# Autodesk Inventor assembly: Leg_Front+Right
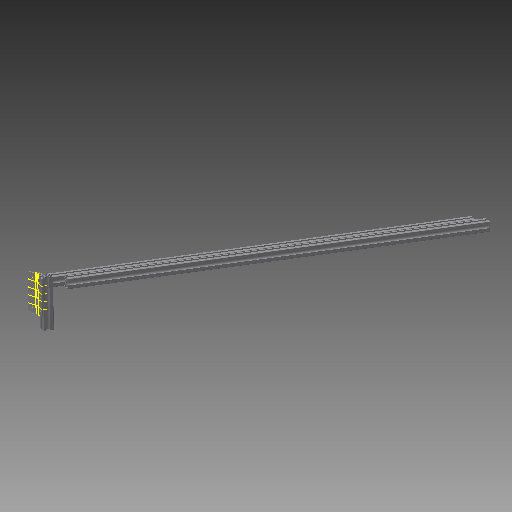
[picture p0: Inventor's stored thumbnail of the model, 512x512]
Saved by Autodesk Inventor 2019 (Build 230136000, 136)
## iProperties
Created: 2019-04-07
Part Number: Leg_Front+Right
Material: 일반
Document SubType Name: Assembly
Designer: hinmo
Author: hinmo
## Documents named in this file (4)
- C:\Users\hinmo\Documents\Inventor\Projects\2019_CapstoneDesign\Leg_Front+Right.iam
- C:\Users\hinmo\Documents\Inventor\Projects\2019_CapstoneDesign\Hinge.iam
- C:\Users\hinmo\Documents\Inventor\Projects\2019_CapstoneDesign\Profile_10.ipt
- C:\Users\hinmo\Documents\Inventor\Projects\2019_CapstoneDesign\Propile_80.ipt
## Components (4 placed, 3 different names)
1. Hinge:1 [sub-assembly] — 플러쉬:1, 메이트:4, 접선:1, 접선:2
2. Profile_10:1 — 플러쉬:1, 플러쉬:2, 메이트:2, 플러쉬:3, 메이트:4, 접선:1, 접선:2
3. Propile_80:1 — 플러쉬:2, 메이트:2, 플러쉬:3, 메이트:3, 플러쉬:4, 플러쉬:5
4. Propile_80:2 — 메이트:3, 플러쉬:4, 플러쉬:5
## Relationships (10: Flush 5, Mate 3, Tangent 2)
- 플러쉬:1 [Flush]: Hinge:1 ↔ Profile_10:1
- 플러쉬:2 [Flush]: Profile_10:1 ↔ Propile_80:1
- 메이트:2 [Mate]: Profile_10:1 ↔ Propile_80:1
- 플러쉬:3 [Flush]: Profile_10:1 ↔ Propile_80:1
- 메이트:3 [Mate]: Propile_80:1 ↔ Propile_80:2
- 플러쉬:4 [Flush]: Propile_80:1 ↔ Propile_80:2
- 플러쉬:5 [Flush] (-20 mm): Propile_80:1 ↔ Propile_80:2
- 메이트:4 [Mate]: Hinge:1 ↔ Profile_10:1
- 접선:1 [Tangent]: Hinge:1 ↔ Profile_10:1
- 접선:2 [Tangent]: Hinge:1 ↔ Profile_10:1
